# Autodesk Inventor assembly: bay con 10 total
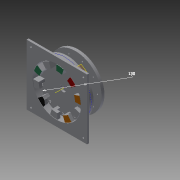
[picture p0: Inventor's stored thumbnail of the model, 180x180]
Saved by Autodesk Inventor 2015 (Build 190159000, 159)
## iProperties
Created: 2014-10-11
Part Number: bay con 10 total
Document SubType Name: Assembly
Designer: ericd_000
Author: ericd_000
## Documents named in this file (4)
- C:\Users\ericd_000\Dropbox\GitHub\initial_cad\eric_cad\bay con 10 total.iam
- C:\Users\ericd_000\Dropbox\GitHub\initial_cad\eric_cad\bayonet container 10.ipt
- C:\Users\ericd_000\Dropbox\GitHub\initial_cad\eric_cad\inner bayonet connector 10.ipt
- C:\Users\ericd_000\Dropbox\GitHub\initial_cad\eric_cad\bay container 10 bottom.ipt
## Components (3 placed, 3 different names)
1. bayonet container 10:1 — Rotational:1, Mate:1
2. inner bayonet connector 10:1 — Rotational:1, Mate:1, Mate:2, Mate:3
3. bay container 10 bottom:1 — Mate:2, Mate:3
## Relationships (4: Mate 3, RevoluteJoint 1)
- Rotational:1 [RevoluteJoint]: bayonet container 10:1 ↔ inner bayonet connector 10:1
- Mate:1: bayonet container 10:1 ↔ inner bayonet connector 10:1
- Mate:2 (20 mm): inner bayonet connector 10:1 ↔ bay container 10 bottom:1
- Mate:3 (20 mm): inner bayonet connector 10:1 ↔ bay container 10 bottom:1
